# Autodesk Inventor assembly: 45degreebracketassembly_MIR
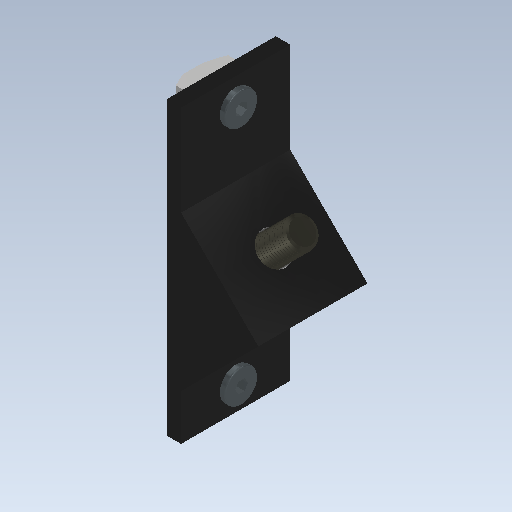
[picture p0: Inventor's stored thumbnail of the model, 512x512]
Saved by Autodesk Inventor 2020.2 (Build 242310000, 310)
## iProperties
Created: 2020-07-25
Part Number: 45degreebracketassembly_MIR
Document SubType Name: Assembly
Designer: JK
Author: JK
## Documents named in this file (5)
- C:\Users\JK\Documents\Inventor\Mesa\45degreebracketassembly_MIR.iam
- C:\Users\JK\Documents\Inventor\Mesa\45degreebracket_MIR.ipt
- C:\Users\JK\Documents\Inventor\Mesa\M5x12BoltFlatHead_MIR.ipt
- C:\Users\JK\Documents\Inventor\Mesa\T_Slot_Nut_Dropin_3030m5ipt_MIR1.ipt
- C:\Users\JK\Documents\Inventor\Mesa\M8x16socketheadbolt_MIR.ipt
## Components (6 placed, 4 different names)
1. 45degreebracket_MIR:1 — Mate:2, Mate:1, Mate:6, Mate:5, Mate:4, Angle:1, Mate:8, Angle:2, Mate:10, Mate:9
2. M5x12BoltFlatHead_MIR:1 — Mate:2, Mate:1, Mate:3
3. M5x12BoltFlatHead_MIR:2 — Mate:6, Mate:5, Mate:7
4. T_Slot_Nut_Dropin_3030m5ipt_MIR1:1 — Mate:4, Angle:1, Mate:3
5. T_Slot_Nut_Dropin_3030m5ipt_MIR1:2 — Mate:8, Angle:2, Mate:7
6. M8x16socketheadbolt_MIR:1 — Mate:10, Mate:9
## Relationships (12: Mate 10, Angle 2)
- Mate:2: 45degreebracket_MIR:1 ↔ M5x12BoltFlatHead_MIR:1
- Mate:1: 45degreebracket_MIR:1 ↔ M5x12BoltFlatHead_MIR:1
- Mate:6: 45degreebracket_MIR:1 ↔ M5x12BoltFlatHead_MIR:2
- Mate:5: 45degreebracket_MIR:1 ↔ M5x12BoltFlatHead_MIR:2
- Mate:4: 45degreebracket_MIR:1 ↔ T_Slot_Nut_Dropin_3030m5ipt_MIR1:1
- Angle:1 (0 deg): 45degreebracket_MIR:1 ↔ T_Slot_Nut_Dropin_3030m5ipt_MIR1:1
- Mate:3: M5x12BoltFlatHead_MIR:1 ↔ T_Slot_Nut_Dropin_3030m5ipt_MIR1:1
- Mate:8: 45degreebracket_MIR:1 ↔ T_Slot_Nut_Dropin_3030m5ipt_MIR1:2
- Angle:2 (0 deg): 45degreebracket_MIR:1 ↔ T_Slot_Nut_Dropin_3030m5ipt_MIR1:2
- Mate:7: M5x12BoltFlatHead_MIR:2 ↔ T_Slot_Nut_Dropin_3030m5ipt_MIR1:2
- Mate:10: 45degreebracket_MIR:1 ↔ M8x16socketheadbolt_MIR:1
- Mate:9: 45degreebracket_MIR:1 ↔ M8x16socketheadbolt_MIR:1
